# Autodesk Inventor assembly: 5su11546kk16
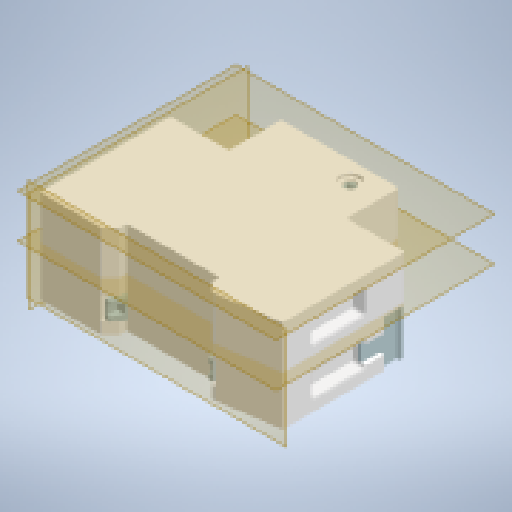
[picture p0: Inventor's stored thumbnail of the model, 512x512]
Saved by Autodesk Inventor 2025.2 (Build 292293000, 293)
## iProperties
Created: 2019-11-22
Part Number: 5su11546kk16
Checked By: TraceParts S.A.
Catalog Web Link: www.traceparts.com
Document SubType Name: Assembly
Designer: TraceParts
Company: TraceParts S.A.
REFERENCE: 5SU11546KK16
DESIGN: FI/LS-protector type A (PSE/SSF), d=70mm IFN 10mA, 10kA, 1+N-pole B 16A
SUPPLIER: SIEMENS
TraceParts.PartNumber: 90-29032019-048374
TraceParts.PartTitle: MCB/RCCB combination
TraceParts.InstanceId: 90-29032019-0483746GXL2JXI8CAKEGWAF8R7PN5LU
TraceParts.PartStatus: Published
TraceParts.PartVersion: 1.0.0
TRACEPARTS: TRACEPARTS
TraceParts.PartLanguage: en
TraceParts.ClassPath: SIEMENS_AUTOMATION:90-29032019-048374
Author: TraceParts
## Documents named in this file (5)
- C:\Users\lucas\OneDrive\Documentos\Documentos\Gustavo\Mozangao\Projeto Base (5140)\Q.E - Braço Robotico\Disjuntor Diferencial\disjuntor_diferencial_999_0001.iam
- C:\Users\lucas\OneDrive\Documentos\Documentos\Gustavo\Mozangao\Projeto Base (5140)\Q.E - Braço Robotico\Disjuntor Diferencial\disjuntor_diferencial_0002_001.ipt
- C:\Users\lucas\OneDrive\Documentos\Documentos\Gustavo\Mozangao\Projeto Base (5140)\Q.E - Braço Robotico\Disjuntor Diferencial\disjuntor_diferencial_0003_001.ipt
- C:\Users\lucas\OneDrive\Documentos\Documentos\Gustavo\Mozangao\Projeto Base (5140)\Q.E - Braço Robotico\Disjuntor Diferencial\disjuntor_diferencial_0004_001.ipt
- C:\Users\lucas\OneDrive\Documentos\Documentos\Gustavo\Mozangao\Projeto Base (5140)\Q.E - Braço Robotico\Disjuntor Diferencial\disjuntor_diferencial_0005_001.ipt
## Components (4 placed, 4 different names)
1. disjuntor_diferencial_0002_001:1 — Simetria:1
2. disjuntor_diferencial_0003_001:1 — Simetria:1
3. disjuntor_diferencial_0004_001:1
4. disjuntor_diferencial_0005_001:1
## Relationships (1: Symmetry 1)
- Simetria:1 [Symmetry]: disjuntor_diferencial_0002_001:1 ↔ disjuntor_diferencial_0003_001:1
